# Autodesk Inventor assembly: SEMIS
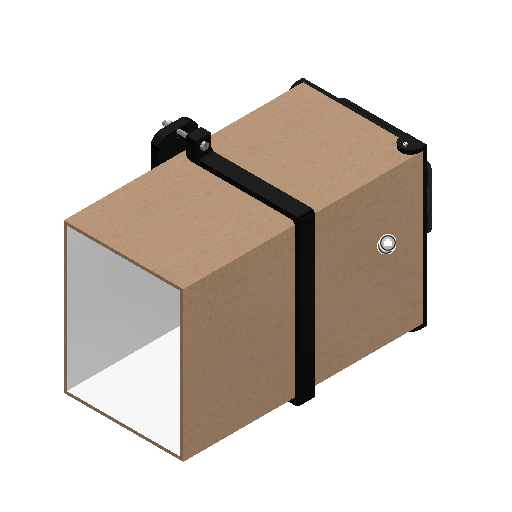
[picture p0: Inventor's stored thumbnail of the model, 512x512]
Saved by Autodesk Inventor 2026.1 (Build 301233000, 233)
## iProperties
Created: 2026-02-27
Part Number: SEMIS
Document SubType Name: Assembly
Designer: aleja
Author: aleja
## Documents named in this file (15)
- C:\Users\aleja\OneDrive\Documentos\Master Studies\Forschungsarbeit\07-3D_modeling\04-SEMIS\SEMIS.iam
- C:\Users\aleja\OneDrive\Documentos\Master Studies\Forschungsarbeit\07-3D_modeling\04-SEMIS\LED_mount.ipt
- C:\Users\aleja\OneDrive\Documentos\Master Studies\Forschungsarbeit\07-3D_modeling\04-SEMIS\FanHolder.ipt
- C:\Users\aleja\OneDrive\Documentos\Master Studies\Forschungsarbeit\07-3D_modeling\04-SEMIS\Reflector.ipt
- C:\Users\aleja\OneDrive\Documentos\Master Studies\Forschungsarbeit\07-3D_modeling\04-SEMIS\Box_clamp_full.ipt
- C:\Users\aleja\OneDrive\Documentos\Master Studies\Forschungsarbeit\07-3D_modeling\04-SEMIS\Power_box.ipt
- C:\Users\aleja\Documents\Inventor\Content Center Files\R2026\en-US\ISO 1207(1)\DIN EN ISO 1207 - M4 x 40.ipt
- C:\Users\aleja\Documents\Inventor\Content Center Files\R2026\en-US\ISO 1207(1)\DIN EN ISO 1207 - M2 x 10.ipt
- C:\Users\aleja\Documents\Inventor\Content Center Files\R2026\en-US\ISO 1207(1)\DIN EN ISO 1207 - M5 x 10.ipt
- C:\Users\aleja\Documents\Inventor\Content Center Files\R2026\en-US\DIN EN ISO 4032\DIN EN ISO 4032 - M4.ipt
- C:\Users\aleja\Documents\Inventor\Content Center Files\R2026\en-US\DIN EN ISO 4032\DIN EN ISO 4032 - M5.ipt
- C:\Users\aleja\Documents\Inventor\Content Center Files\R2026\en-US\DIN EN ISO 4032\DIN EN ISO 4032 - M2.ipt
- C:\Users\aleja\OneDrive\Documentos\Master Studies\Forschungsarbeit\07-3D_modeling\04-SEMIS\RedLEDArray.ipt
- C:\Users\aleja\OneDrive\Documentos\Master Studies\Forschungsarbeit\07-3D_modeling\04-SEMIS\fan.ipt
- C:\Users\aleja\OneDrive\Documentos\Master Studies\Forschungsarbeit\07-3D_modeling\04-SEMIS\whiteLEDArray.ipt
## Components (49 placed, 14 different names)
1. LED_mount:1 — Planar:1, Mate:1, Mate:2, Flush:1, Mate:7, Mate:8, Mate:9, Mate:10, Mate:11, Mate:12, Mate:13, Mate:14, Mate:17, Insert:2, Insert:3, Insert:4, Insert:5, Insert:6, Insert:7, Insert:8, Insert:9, Mate:30, Mate:31, Mate:32, Mate:33, Mate:34, Mate:35, Mate:36, Mate:38, Mate:40, Mate:41, Mate:42, Mate:43, Insert:10, Insert:11, Insert:12, Insert:13, Mate:46, Mate:47, Mate:50, Mate:51, Mate:52
2. FanHolder:1 — Planar:1, Mate:1, Mate:2, Mate:5, Mate:48
3. Reflector:1 — Flush:1, Rigid:1, Mate:3, Mate:23, Mate:25, Mate:27, Mate:29, Mate:30, Mate:36
4. Box_clamp_full:1 — Rigid:1, Mate:4, Mate:15, Mate:16, Mate:18, Mate:19
5. Power_box:1 — Mate:3, Mate:4, Insert:1, Mate:21
6. DIN EN ISO 1207 M4 x 40:3 — Mate:15, Mate:16
7. DIN EN ISO 1207 M4 x 40:4 — Mate:18, Mate:19, Mate:20
8. DIN EN ISO 1207 M2 x 10:1 — Mate:13, Mate:37, Mate:44
9. DIN EN ISO 1207 M2 x 10:2 — Mate:8, Mate:9, Mate:22
10. DIN EN ISO 1207 M2 x 10:3 — Mate:17, Mate:39, Mate:45
11. DIN EN ISO 1207 M2 x 10:4 — Mate:12, Mate:24, Mate:33
12. DIN EN ISO 1207 M2 x 10:5 — Mate:11, Mate:26, Mate:31
13. DIN EN ISO 1207 M2 x 10:6 — Mate:10, Mate:28, Mate:32
14. DIN EN ISO 4032 M4:1 — Insert:1
15. DIN EN ISO 4032 M4:2 — Mate:20, Mate:21
16. DIN EN ISO 4032 M5:1 — Insert:2
17. DIN EN ISO 4032 M5:2 — Insert:3
18. DIN EN ISO 4032 M5:3 — Insert:4
19. DIN EN ISO 4032 M5:4 — Insert:5
20. DIN EN ISO 4032 M5:5 — Insert:6
21. DIN EN ISO 4032 M5:6 — Insert:7
22. DIN EN ISO 4032 M5:7 — Insert:8
23. DIN EN ISO 4032 M5:8 — Insert:9
24. DIN EN ISO 4032 M2:1 — Mate:22, Mate:23
25. DIN EN ISO 4032 M2:2 — Mate:24, Mate:25
26. DIN EN ISO 4032 M2:3 — Mate:26, Mate:27
27. DIN EN ISO 4032 M2:4 — Mate:28, Mate:29
28. DIN EN ISO 4032 M2:5 — Mate:37, Mate:38
29. DIN EN ISO 4032 M2:6 — Mate:39, Mate:40
30. RedLEDArray:1 — Mate:41, Mate:42, Mate:43, Mate:44, Mate:45
31. DIN EN ISO 4032 M4:3 — Insert:10
32. DIN EN ISO 4032 M4:4 — Insert:11
33. DIN EN ISO 4032 M4:5 — Insert:12
34. DIN EN ISO 4032 M4:6 — Insert:13
35. fan:1 — Mate:46, Mate:47, Mate:48, Mate:49
36. DIN EN ISO 1207 M4 x 40:2 — Mate:5, Mate:49
37. DIN EN ISO 1207 M4 x 40:7
38. DIN EN ISO 1207 M4 x 40:8
39. DIN EN ISO 1207 M4 x 40:9
40. DIN EN ISO 1207 M5 x 10:3 — Mate:7
41. DIN EN ISO 1207 M5 x 10:9 — Mate:35
42. DIN EN ISO 1207 M5 x 10:10
43. DIN EN ISO 1207 M5 x 10:11
44. DIN EN ISO 1207 M5 x 10:4 — Mate:14
45. DIN EN ISO 1207 M5 x 10:12
46. DIN EN ISO 1207 M5 x 10:13 — Mate:34
47. DIN EN ISO 1207 M5 x 10:14
48. whiteLEDArray:1 — Mate:50, Mate:51, Mate:52
49. whiteLEDArray:2
## Component patterns: (4 elements, first: DIN EN ISO 1207 M4 x 40:2), (4 elements, first: DIN EN ISO 1207 M5 x 10:3), (4 elements, first: DIN EN ISO 1207 M5 x 10:4), (2 elements, first: whiteLEDArray:1)
## Relationships (67: Mate 51, Insert 13, PlanarJoint 1, Flush 1, WeldJoint 1)
- Planar:1: LED_mount:1 ↔ FanHolder:1
- Mate:1: LED_mount:1 ↔ FanHolder:1
- Mate:2: LED_mount:1 ↔ FanHolder:1
- Flush:1: LED_mount:1 ↔ Reflector:1
- Rigid:1 [WeldJoint]: Reflector:1 ↔ Box_clamp_full:1
- Mate:3 (5 mm): Reflector:1 ↔ Power_box:1
- Mate:4: Box_clamp_full:1 ↔ Power_box:1
- Mate:5: FanHolder:1 ↔ DIN EN ISO 1207 M4 x 40:2
- Mate:7: LED_mount:1 ↔ DIN EN ISO 1207 M5 x 10:3
- Mate:8: LED_mount:1 ↔ DIN EN ISO 1207 M2 x 10:2
- Mate:9: LED_mount:1 ↔ DIN EN ISO 1207 M2 x 10:2
- Mate:10: LED_mount:1 ↔ DIN EN ISO 1207 M2 x 10:6
- Mate:11: LED_mount:1 ↔ DIN EN ISO 1207 M2 x 10:5
- Mate:12: LED_mount:1 ↔ DIN EN ISO 1207 M2 x 10:4
- Mate:13: LED_mount:1 ↔ DIN EN ISO 1207 M2 x 10:1
- Mate:14: LED_mount:1 ↔ DIN EN ISO 1207 M5 x 10:4
- Mate:15: Box_clamp_full:1 ↔ DIN EN ISO 1207 M4 x 40:3
- Mate:16: Box_clamp_full:1 ↔ DIN EN ISO 1207 M4 x 40:3
- Mate:17: LED_mount:1 ↔ DIN EN ISO 1207 M2 x 10:3
- Mate:18: Box_clamp_full:1 ↔ DIN EN ISO 1207 M4 x 40:4
- Mate:19: Box_clamp_full:1 ↔ DIN EN ISO 1207 M4 x 40:4
- Insert:1: Power_box:1 ↔ DIN EN ISO 4032 M4:1
- Mate:20: DIN EN ISO 1207 M4 x 40:4 ↔ DIN EN ISO 4032 M4:2
- Mate:21: Power_box:1 ↔ DIN EN ISO 4032 M4:2
- Insert:2: LED_mount:1 ↔ DIN EN ISO 4032 M5:1
- Insert:3: LED_mount:1 ↔ DIN EN ISO 4032 M5:2
- Insert:4: LED_mount:1 ↔ DIN EN ISO 4032 M5:3
- Insert:5: LED_mount:1 ↔ DIN EN ISO 4032 M5:4
- Insert:6: LED_mount:1 ↔ DIN EN ISO 4032 M5:5
- Insert:7: LED_mount:1 ↔ DIN EN ISO 4032 M5:6
- Insert:8: LED_mount:1 ↔ DIN EN ISO 4032 M5:7
- Insert:9: LED_mount:1 ↔ DIN EN ISO 4032 M5:8
- Mate:22: DIN EN ISO 1207 M2 x 10:2 ↔ DIN EN ISO 4032 M2:1
- Mate:23: Reflector:1 ↔ DIN EN ISO 4032 M2:1
- Mate:24: DIN EN ISO 1207 M2 x 10:4 ↔ DIN EN ISO 4032 M2:2
- Mate:25: Reflector:1 ↔ DIN EN ISO 4032 M2:2
- Mate:26: DIN EN ISO 1207 M2 x 10:5 ↔ DIN EN ISO 4032 M2:3
- Mate:27: Reflector:1 ↔ DIN EN ISO 4032 M2:3
- Mate:28: DIN EN ISO 1207 M2 x 10:6 ↔ DIN EN ISO 4032 M2:4
- Mate:29: Reflector:1 ↔ DIN EN ISO 4032 M2:4
- Mate:30: LED_mount:1 ↔ Reflector:1
- Mate:31: LED_mount:1 ↔ DIN EN ISO 1207 M2 x 10:5
- Mate:32: LED_mount:1 ↔ DIN EN ISO 1207 M2 x 10:6
- Mate:33: LED_mount:1 ↔ DIN EN ISO 1207 M2 x 10:4
- Mate:34: LED_mount:1 ↔ DIN EN ISO 1207 M5 x 10:13
- Mate:35: LED_mount:1 ↔ DIN EN ISO 1207 M5 x 10:9
- Mate:36: LED_mount:1 ↔ Reflector:1
- Mate:37: DIN EN ISO 1207 M2 x 10:1 ↔ DIN EN ISO 4032 M2:5
- Mate:38: LED_mount:1 ↔ DIN EN ISO 4032 M2:5
- Mate:39: DIN EN ISO 1207 M2 x 10:3 ↔ DIN EN ISO 4032 M2:6
- Mate:40: LED_mount:1 ↔ DIN EN ISO 4032 M2:6
- Mate:41: LED_mount:1 ↔ RedLEDArray:1
- Mate:42: LED_mount:1 ↔ RedLEDArray:1
- Mate:43: LED_mount:1 ↔ RedLEDArray:1
- Mate:44: DIN EN ISO 1207 M2 x 10:1 ↔ RedLEDArray:1
- Mate:45: DIN EN ISO 1207 M2 x 10:3 ↔ RedLEDArray:1
- Insert:10: LED_mount:1 ↔ DIN EN ISO 4032 M4:3
- Insert:11: LED_mount:1 ↔ DIN EN ISO 4032 M4:4
- Insert:12: LED_mount:1 ↔ DIN EN ISO 4032 M4:5
- Insert:13: LED_mount:1 ↔ DIN EN ISO 4032 M4:6
- Mate:46: LED_mount:1 ↔ fan:1
- Mate:47: LED_mount:1 ↔ fan:1
- Mate:48: FanHolder:1 ↔ fan:1
- Mate:49: fan:1 ↔ DIN EN ISO 1207 M4 x 40:2
- Mate:50: LED_mount:1 ↔ whiteLEDArray:1
- Mate:51: LED_mount:1 ↔ whiteLEDArray:1
- Mate:52: LED_mount:1 ↔ whiteLEDArray:1
## Named parameters: Finish3_Area = 1387.91
note: some values were not read from the file. Shown as the stored number, unit unknown: "Finish3_Area".
